# Autodesk Inventor assembly: TWambat Side
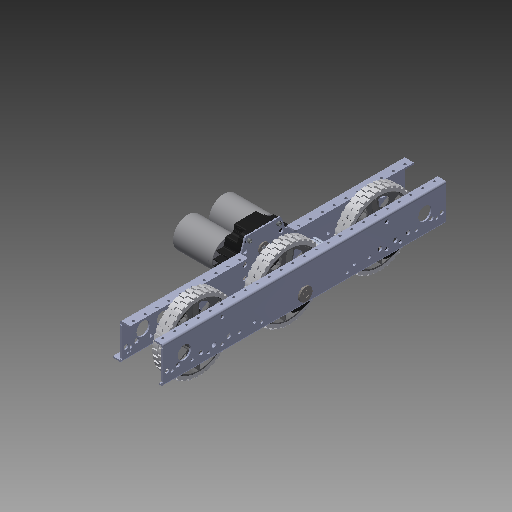
[picture p0: Inventor's stored thumbnail of the model, 512x512]
Saved by Autodesk Inventor 2019 (Build 230136000, 136)
## iProperties
Created: 2019-12-10
Part Number: TWambat Side
Document SubType Name: Assembly
Designer: james
Author: james
## Documents named in this file (7)
- F:\JimsRobot\FIRSTRobots\Design\TWambat\TWambat Side.iam
- F:\JimsRobot\FIRSTRobots\Design\TWambat\TWambat Side Frame.iam
- F:\JimsRobot\FIRSTRobots\Design\Library\AndyMark\6 HiGrip with bearings, pulleys and spacers.iam
- F:\JimsRobot\FIRSTRobots\Design\Library\AndyMark\6 HiGrip with hub and double pulley.iam
- F:\JimsRobot\FIRSTRobots\Design\Library\AndyMark\FR8ZZ Hex Bearing.ipt
- F:\JimsRobot\FIRSTRobots\Design\Library\AndyMark\am-2598_107 2016 KOP Toughbox Mini.iam
- F:\JimsRobot\FIRSTRobots\Design\Library\AndyMark\Mini_CIM_Motor_217-3371.ipt
## Components (8 placed, 6 different names)
1. TWambat Side Frame:1 [sub-assembly] — Mate:1, Mate:2, Mate:3, Mate:4, Mate:5, Mate:6, Mate:10, Mate:11, Mate:12
2. 6 HiGrip with bearings, pulleys and spacers:1 [sub-assembly] — Mate:1, Mate:2
3. 6 HiGrip with bearings, pulleys and spacers:2 [sub-assembly] — Mate:3, Mate:4
4. 6 HiGrip with hub and double pulley:1 [sub-assembly] — Mate:7, Mate:8
5. FR8ZZ Hex Bearing:1 — Mate:5, Mate:6, Mate:7, Mate:8
6. am-2598_107 2016 KOP Toughbox Mini:1 [sub-assembly] — Mate:10, Mate:11, Mate:12, Mate:13, Mate:14, Mate:15, Mate:16
7. Mini_CIM_Motor_217-3371:1 — Mate:14, Mate:15
8. Mini_CIM_Motor_217-3371:2 — Mate:13, Mate:16
## Relationships (15: Mate 15)
- Mate:1: TWambat Side Frame:1 ↔ 6 HiGrip with bearings, pulleys and spacers:1
- Mate:2: TWambat Side Frame:1 ↔ 6 HiGrip with bearings, pulleys and spacers:1
- Mate:3: TWambat Side Frame:1 ↔ 6 HiGrip with bearings, pulleys and spacers:2
- Mate:4: TWambat Side Frame:1 ↔ 6 HiGrip with bearings, pulleys and spacers:2
- Mate:5: TWambat Side Frame:1 ↔ FR8ZZ Hex Bearing:1
- Mate:6: TWambat Side Frame:1 ↔ FR8ZZ Hex Bearing:1
- Mate:7: 6 HiGrip with hub and double pulley:1 ↔ FR8ZZ Hex Bearing:1
- Mate:8: 6 HiGrip with hub and double pulley:1 ↔ FR8ZZ Hex Bearing:1
- Mate:10: TWambat Side Frame:1 ↔ am-2598_107 2016 KOP Toughbox Mini:1
- Mate:11: TWambat Side Frame:1 ↔ am-2598_107 2016 KOP Toughbox Mini:1
- Mate:12: TWambat Side Frame:1 ↔ am-2598_107 2016 KOP Toughbox Mini:1
- Mate:13: am-2598_107 2016 KOP Toughbox Mini:1 ↔ Mini_CIM_Motor_217-3371:2
- Mate:14: am-2598_107 2016 KOP Toughbox Mini:1 ↔ Mini_CIM_Motor_217-3371:1
- Mate:15: am-2598_107 2016 KOP Toughbox Mini:1 ↔ Mini_CIM_Motor_217-3371:1
- Mate:16: am-2598_107 2016 KOP Toughbox Mini:1 ↔ Mini_CIM_Motor_217-3371:2
